# Autodesk Inventor assembly: Rail_AssemblyV2_0
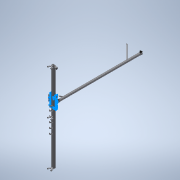
[picture p0: Inventor's stored thumbnail of the model, 180x180]
Saved by Autodesk Inventor 2021 (Build 250183000, 183)
## iProperties
Created: 2021-01-25
Part Number: Rail_AssemblyV2_0
Document SubType Name: Assembly
Designer: Jorian Brusind
Mass: 3786.54 g
Surface Area: 19508.5 cm^2
Volume: 2323.9 cm^3
Density: 1.62939 g/cm^3
Author: Jorian Brusind
## Documents named in this file (30)
- C:\Users\Jorian Brusind\Documents\GitHub\PersonalProjects\HyperRail\Inventor Files\Rail_AssemblyV2_0.iam
- C:\Users\Jorian Brusind\Documents\GitHub\PersonalProjects\Inventor Projects\Useful models\NEMA_Steppers\NEMA23\23HS8430B.ipt
- C:\Users\Jorian Brusind\Documents\GitHub\PersonalProjects\HyperRail\Inventor Files\2804S_NEMA2115_1Gearbox.ipt
- C:\Users\Jorian Brusind\Documents\GitHub\PersonalProjects\HyperRail\PCB Files\Integrated Stepper Motor Driver\ExportSTEP\Main.iam
- C:\Users\Jorian Brusind\Documents\GitHub\PersonalProjects\HyperRail\Inventor Files\NEMA23_Shroud.ipt
- C:\Users\Jorian Brusind\Documents\GitHub\PersonalProjects\Inventor Projects\Useful models\8020_Sets\IPT_20_Series\IPT_20_Series\20-4040_2m.ipt
- C:\Users\Jorian Brusind\Documents\GitHub\PersonalProjects\HyperRail\Inventor Files\98952A059_ALUM MALE-FEM THRDED HEX STANDOFF.ipt
- C:\Users\Jorian Brusind\Documents\GitHub\PersonalProjects\HyperRail\Inventor Files\95783A039_NYLON 6-6 MALE-FEM THRDED HEX STANDOFF.ipt
- C:\Users\Jorian Brusind\Documents\GitHub\PersonalProjects\HyperRail\Inventor Files\Integrated_Stepper_NEMA23_Mount.ipt
- C:\Users\Jorian Brusind\Documents\GitHub\PersonalProjects\Inventor Projects\Useful models\8020_Sets\IPT_40_Series\Extra_40_Series\HFS5-4060-4000\HFS5-4060-2125.ipt
- C:\Users\Jorian Brusind\Documents\GitHub\PersonalProjects\Inventor Projects\Useful models\8020_Sets\AIS2018\20-2568_d.iam
- C:\Users\Jorian Brusind\Documents\GitHub\PersonalProjects\HyperRail\Inventor Files\5mm_bore_10mm_width_idlepulley.ipt
- C:\Users\Jorian Brusind\Documents\GitHub\PersonalProjects\HyperRail\Inventor Files\Tape_Belt_Layer.ipt
- C:\Users\Jorian Brusind\Documents\GitHub\PersonalProjects\HyperRail\Inventor Files\SDP_sdpsi_a_6a55m028df0912\SDP_sdpsi_a_6a55m028df0912.ipt
- C:\Users\Jorian Brusind\Documents\GitHub\PersonalProjects\HyperRail\Inventor Files\SDP_sdpsi_a_6r25mc250\SDP_sdpsi_a_6r25mc1000.ipt
- C:\Users\Jorian Brusind\Documents\GitHub\PersonalProjects\HyperRail\Inventor Files\Cable_Guide_Holder.ipt
- C:\Users\Jorian Brusind\Documents\GitHub\PersonalProjects\HyperRail\Inventor Files\Carriage_Assembly.iam
- C:\Users\Jorian Brusind\Documents\GitHub\PersonalProjects\HyperRail\Inventor Files\NEMA23_StepperonlineMount.ipt
- C:\Users\Jorian Brusind\Documents\GitHub\PersonalProjects\HyperRail\Inventor Files\59145_Sensor.ipt
- C:\Users\Jorian Brusind\Documents\GitHub\PersonalProjects\HyperRail\Inventor Files\RightAngle_SideBracket.ipt
- C:\Users\Jorian Brusind\Documents\GitHub\PersonalProjects\HyperRail\Inventor Files\RightAngle_PulleySupport.ipt
- C:\Users\Jorian Brusind\Documents\GitHub\PersonalProjects\HyperRail\Inventor Files\MagnetHolder.ipt
- C:\Users\Jorian Brusind\Documents\GitHub\PersonalProjects\HyperRail\Inventor Files\MagnetActuatorHolder.ipt
- C:\Users\Jorian Brusind\Documents\GitHub\PersonalProjects\HyperRail\Inventor Files\59145_Actuator.ipt
- C:\Users\Jorian Brusind\Documents\GitHub\PersonalProjects\HyperRail\Inventor Files\Bottom_Foot_Assembly.iam
- C:\Users\Jorian Brusind\Documents\GitHub\PersonalProjects\Inventor Projects\Useful models\Metric bolt\Bolt M5 8mm.ipt
- C:\Users\Jorian Brusind\Documents\GitHub\PersonalProjects\Inventor Projects\Useful models\Metric bolt\Bolt M5 12mm.ipt
- C:\Users\Jorian Brusind\Documents\GitHub\PersonalProjects\Inventor Projects\Useful models\Metric bolt\Bolt M5 25mm.ipt
- C:\Users\Jorian Brusind\Documents\GitHub\PersonalProjects\Inventor Projects\Useful models\Metric bolt\Bolt M4 10mm.ipt
- C:\Users\Jorian Brusind\Documents\GitHub\PersonalProjects\HyperRail\Inventor Files\RightAngle_Bracket_60mm.ipt
## Components (79 placed, 29 different names)
1. 23HS8430B:1 — Mate:127, Angle:3, Mate:158, Mate:177, Mate:179, Mate:180, Mate:181, Mate:182, Mate:183, Mate:184, Mate:185, Mate:264, Mate:265, Mate:295, Angle:5, Angle:6
2. 2804S_NEMA2115_1Gearbox:1 — Mate:127, Angle:3, Mate:158, Flush:86, Mate:336, Flush:126, Mate:370, Mate:371
3. Main:1 [sub-assembly] — Mate:291, Mate:292, Mate:293
4. 20-4040_2m:2 — Flush:123, Mate:322, Mate:323, Mate:354, Flush:143, Flush:156, Mate:375, Flush:158, Mate:377, Mate:378, Flush:160, Flush:161, Flush:163, Flush:189, Mate:420, Flush:190, Mate:474
5. NEMA23_Shroud:1 — Mate:264, Mate:265, Flush:86, Angle:7, Mate:452, Mate:453, Mate:454, Mate:455, Mate:456, Mate:457, Mate:458, Mate:459
6. 98952A059_ALUM MALE-FEM THRDED HEX STANDOFF:1 — Mate:180, Mate:181, Mate:186, Mate:191
7. 98952A059_ALUM MALE-FEM THRDED HEX STANDOFF:2 — Mate:184, Mate:185, Mate:189, Mate:192
8. 98952A059_ALUM MALE-FEM THRDED HEX STANDOFF:3 — Mate:177, Mate:179, Mate:187, Mate:190
9. 98952A059_ALUM MALE-FEM THRDED HEX STANDOFF:4 — Mate:182, Mate:183, Mate:188, Mate:193
10. 95783A039_NYLON 6-6 MALE-FEM THRDED HEX STANDOFF:1 — Mate:188, Mate:193
11. 95783A039_NYLON 6-6 MALE-FEM THRDED HEX STANDOFF:2 — Mate:186, Mate:191, Mate:369
12. 95783A039_NYLON 6-6 MALE-FEM THRDED HEX STANDOFF:3 — Mate:187, Mate:190
13. 95783A039_NYLON 6-6 MALE-FEM THRDED HEX STANDOFF:4 — Mate:189, Mate:192
14. HFS5-4060-2125:1 — Mate:277, Mate:278, Mate:279, Mate:280, Mate:332, Mate:333, Mate:344, Flush:132, Flush:133, Mate:353, Mate:366, Mate:413, Flush:179, Mate:418, Mate:428, Flush:195, Flush:196, Mate:431, Flush:197, Flush:198, Mate:494, Mate:495
15. Integrated_Stepper_NEMA23_Mount:1 — Mate:291, Mate:292, Mate:293, Mate:295, Mate:360, Mate:361, Mate:362, Mate:363, Mate:364, Mate:369, Angle:5, Angle:6
16. 20-2568_d:1 [sub-assembly] — Flush:123, Mate:322, Mate:323
17. 5mm_bore_10mm_width_idlepulley:2 — Mate:421, Mate:422, Mate:446, Mate:447
18. Tape_Belt_Layer:1 — Mate:332, Mate:333
19. SDP_sdpsi_a_6a55m028df0912:1 — Mate:336, Flush:126, Flush:191
20. SDP_sdpsi_a_6r25mc1000:1 — Flush:130, Mate:343, Flush:131, Mate:344, Flush:132, Flush:133
21. SDP_sdpsi_a_6r25mc1000:2 — Flush:130, Mate:343, Flush:131
22. Carriage_Assembly:1 [sub-assembly] — Mate:353, Mate:354, Flush:143, Mate:366, Mate:372, Flush:153, Flush:157, Flush:159, Flush:189, Flush:191, Mate:427, Flush:193, Flush:194, Mate:460, Mate:463, Mate:475, Mate:477, Mate:494, Mate:495
23. 98952A059_ALUM MALE-FEM THRDED HEX STANDOFF:5 — Mate:360, Flush:151, Flush:152
24. 98952A059_ALUM MALE-FEM THRDED HEX STANDOFF:6 — Mate:361, Flush:152
25. 98952A059_ALUM MALE-FEM THRDED HEX STANDOFF:7 — Mate:362, Mate:364, Flush:150, Flush:151
26. 98952A059_ALUM MALE-FEM THRDED HEX STANDOFF:8 — Mate:363, Flush:150
27. NEMA23_StepperonlineMount:1 — Mate:370, Mate:371, Angle:7, Mate:372, Flush:153, Mate:461, Mate:462, Mate:464, Mate:465
28. 59145_Sensor:1 — Mate:425, Mate:426, Angle:8
29. RightAngle_SideBracket:1 — Mate:375, Flush:158, Flush:159, Mate:476, Mate:478, Mate:479, Mate:480, Mate:481, Mate:482, Mate:483, Mate:484, Mate:485
30. RightAngle_SideBracket:2 — Flush:156, Flush:157, Mate:473, Mate:474, Mate:486, Mate:487, Mate:488, Mate:489, Mate:490, Mate:491, Mate:492, Mate:493
31. RightAngle_SideBracket:3 — Mate:378, Flush:160, Flush:162, Flush:163, Mate:438, Mate:439, Mate:440, Mate:441, Mate:442, Mate:443
32. RightAngle_SideBracket:4 — Mate:377, Flush:161, Flush:162, Mate:432, Mate:433, Mate:434, Mate:435, Mate:436, Mate:437
33. Cable_Guide_Holder:1 — Mate:413, Flush:179, Flush:188, Mate:419
34. Cable_Guide_Holder:2 — Mate:414, Flush:180, Flush:181
35. Cable_Guide_Holder:3 — Mate:414, Flush:180, Flush:181, Flush:182, Flush:183, Flush:186, Flush:187, Mate:415
36. Cable_Guide_Holder:4 — Flush:182, Flush:187, Mate:415, Mate:416
37. Cable_Guide_Holder:5 — Flush:183, Flush:184, Flush:185, Flush:186, Mate:417, Mate:418, Flush:188
38. Cable_Guide_Holder:6 — Flush:184, Flush:185, Mate:416, Mate:417, Mate:419
39. RightAngle_PulleySupport:1 — Mate:420, Flush:190, Mate:421, Mate:422, Mate:444, Mate:445
40. MagnetHolder:1 — Mate:425, Mate:426, Mate:427, Flush:193, Angle:8, Flush:194
41. MagnetActuatorHolder:1 — Mate:428, Flush:195, Flush:196, Mate:429, Angle:9, Mate:430, Mate:448, Mate:449, Mate:450, Mate:451
42. 59145_Actuator:1 — Mate:429, Angle:9, Mate:430
43. Bolt M5 8mm:1 — Mate:434, Flush:199, Flush:200, Flush:201, Flush:202, Mate:437
44. Bolt M5 8mm:2 — Mate:432, Flush:201
45. Bolt M5 8mm:3 — Mate:435, Flush:199
46. Bolt M5 8mm:4 — Mate:433, Flush:202
47. Bolt M5 8mm:5 — Mate:442, Flush:206
48. Bolt M5 8mm:6 — Mate:440, Flush:204
49. Bolt M5 8mm:7 — Mate:439, Flush:203, Flush:204, Flush:205, Flush:206, Mate:443
50. Bolt M5 8mm:8 — Mate:438, Flush:203
51. Bolt M5 8mm:9 — Mate:441, Flush:205
52. Bolt M5 8mm:10 — Mate:436, Flush:200
53. Bolt M5 12mm:1 — Mate:444, Mate:445
54. Bolt M5 25mm:1 — Mate:446, Mate:447
55. Bolt M5 12mm:2 — Mate:448, Mate:450
56. Bolt M5 12mm:3 — Mate:449, Mate:451
57. Bolt M4 10mm:1 — Mate:453, Mate:456
58. Bolt M4 10mm:2 — Mate:454, Mate:459
59. Bolt M4 10mm:3 — Mate:455, Mate:458
60. Bolt M4 10mm:4 — Mate:452, Mate:457
61. RightAngle_Bracket_60mm:1 — Mate:460, Mate:461, Mate:464, Mate:468, Mate:469, Mate:470, Mate:471
62. RightAngle_Bracket_60mm:2 — Mate:462, Mate:463, Mate:465, Mate:466, Mate:467, Mate:472
63. Bolt M5 12mm:4 — Mate:469, Mate:471
64. Bolt M5 12mm:5 — Mate:468, Mate:470
65. Bolt M5 12mm:6 — Mate:467
66. Bolt M5 12mm:7 — Mate:466, Mate:472
67. Bolt M5 12mm:8 — Mate:473, Mate:475
68. Bolt M5 12mm:9 — Mate:476, Mate:477
69. Bolt M5 8mm:11 — Mate:478, Mate:483
70. Bolt M5 8mm:12 — Mate:479, Mate:482
71. Bolt M5 8mm:13 — Mate:480, Mate:484
72. Bolt M5 8mm:14 — Mate:481, Mate:485
73. Bolt M5 8mm:15 — Mate:486, Mate:492
74. Bolt M5 8mm:16 — Mate:489, Mate:490
75. Bolt M5 8mm:17 — Mate:487, Mate:491
76. Bolt M5 8mm:18 — Mate:488, Mate:493
77. Bottom_Foot_Assembly:1 [sub-assembly] — Mate:431, Flush:197, Flush:198
78. Bottom_Foot_Assembly:2 [sub-assembly]
79. Bottom_Foot_Assembly:3 [sub-assembly]
## Component patterns: (3 elements, first: Bottom_Foot_Assembly:1)
## Relationships (184: Mate 131, Flush 47, Angle 6)
- Mate:127: 23HS8430B:1 ↔ 2804S_NEMA2115_1Gearbox:1
- Angle:3 (0 deg): 23HS8430B:1 ↔ 2804S_NEMA2115_1Gearbox:1
- Mate:158: 23HS8430B:1 ↔ 2804S_NEMA2115_1Gearbox:1
- Mate:177: 23HS8430B:1 ↔ 98952A059_ALUM MALE-FEM THRDED HEX STANDOFF:3
- Mate:179: 23HS8430B:1 ↔ 98952A059_ALUM MALE-FEM THRDED HEX STANDOFF:3
- Mate:180: 23HS8430B:1 ↔ 98952A059_ALUM MALE-FEM THRDED HEX STANDOFF:1
- Mate:181: 23HS8430B:1 ↔ 98952A059_ALUM MALE-FEM THRDED HEX STANDOFF:1
- Mate:182: 23HS8430B:1 ↔ 98952A059_ALUM MALE-FEM THRDED HEX STANDOFF:4
- Mate:183: 23HS8430B:1 ↔ 98952A059_ALUM MALE-FEM THRDED HEX STANDOFF:4
- Mate:184: 23HS8430B:1 ↔ 98952A059_ALUM MALE-FEM THRDED HEX STANDOFF:2
- Mate:185: 23HS8430B:1 ↔ 98952A059_ALUM MALE-FEM THRDED HEX STANDOFF:2
- Mate:186: 98952A059_ALUM MALE-FEM THRDED HEX STANDOFF:1 ↔ 95783A039_NYLON 6-6 MALE-FEM THRDED HEX STANDOFF:2
- Mate:187: 98952A059_ALUM MALE-FEM THRDED HEX STANDOFF:3 ↔ 95783A039_NYLON 6-6 MALE-FEM THRDED HEX STANDOFF:3
- Mate:188: 98952A059_ALUM MALE-FEM THRDED HEX STANDOFF:4 ↔ 95783A039_NYLON 6-6 MALE-FEM THRDED HEX STANDOFF:1
- Mate:189: 98952A059_ALUM MALE-FEM THRDED HEX STANDOFF:2 ↔ 95783A039_NYLON 6-6 MALE-FEM THRDED HEX STANDOFF:4
- Mate:190: 98952A059_ALUM MALE-FEM THRDED HEX STANDOFF:3 ↔ 95783A039_NYLON 6-6 MALE-FEM THRDED HEX STANDOFF:3
- Mate:191: 98952A059_ALUM MALE-FEM THRDED HEX STANDOFF:1 ↔ 95783A039_NYLON 6-6 MALE-FEM THRDED HEX STANDOFF:2
- Mate:192: 98952A059_ALUM MALE-FEM THRDED HEX STANDOFF:2 ↔ 95783A039_NYLON 6-6 MALE-FEM THRDED HEX STANDOFF:4
- Mate:193: 98952A059_ALUM MALE-FEM THRDED HEX STANDOFF:4 ↔ 95783A039_NYLON 6-6 MALE-FEM THRDED HEX STANDOFF:1
- Mate:264 (1 mm): 23HS8430B:1 ↔ NEMA23_Shroud:1
- Mate:265 (1 mm): 23HS8430B:1 ↔ NEMA23_Shroud:1
- Flush:86: 2804S_NEMA2115_1Gearbox:1 ↔ NEMA23_Shroud:1
- Mate:277: HFS5-4060-2125:1
- Mate:278: HFS5-4060-2125:1
- Mate:279: HFS5-4060-2125:1
- Mate:280: HFS5-4060-2125:1
- Mate:291: Main:1 ↔ Integrated_Stepper_NEMA23_Mount:1
- Mate:292: Main:1 ↔ Integrated_Stepper_NEMA23_Mount:1
- Mate:293: Main:1 ↔ Integrated_Stepper_NEMA23_Mount:1
- Mate:295: 23HS8430B:1 ↔ Integrated_Stepper_NEMA23_Mount:1
- Flush:123: 20-4040_2m:2 ↔ 20-2568_d:1
- Mate:322 (-2 mm): 20-4040_2m:2 ↔ 20-2568_d:1
- Mate:323: 20-4040_2m:2 ↔ 20-2568_d:1
- Mate:332: HFS5-4060-2125:1 ↔ Tape_Belt_Layer:1
- Mate:333 (1 mm): HFS5-4060-2125:1 ↔ Tape_Belt_Layer:1
- Mate:336: 2804S_NEMA2115_1Gearbox:1 ↔ SDP_sdpsi_a_6a55m028df0912:1
- Flush:126: 2804S_NEMA2115_1Gearbox:1 ↔ SDP_sdpsi_a_6a55m028df0912:1
- Flush:130: SDP_sdpsi_a_6r25mc1000:1 ↔ SDP_sdpsi_a_6r25mc1000:2
- Mate:343: SDP_sdpsi_a_6r25mc1000:1 ↔ SDP_sdpsi_a_6r25mc1000:2
- Flush:131: SDP_sdpsi_a_6r25mc1000:1 ↔ SDP_sdpsi_a_6r25mc1000:2
- Mate:344 (1 mm): HFS5-4060-2125:1 ↔ SDP_sdpsi_a_6r25mc1000:1
- Flush:132: HFS5-4060-2125:1 ↔ SDP_sdpsi_a_6r25mc1000:1
- Flush:133: HFS5-4060-2125:1 ↔ SDP_sdpsi_a_6r25mc1000:1
- Mate:353 (6 mm): HFS5-4060-2125:1 ↔ Carriage_Assembly:1
- Mate:354: 20-4040_2m:2 ↔ Carriage_Assembly:1
- Flush:143: 20-4040_2m:2 ↔ Carriage_Assembly:1
- Mate:360: Integrated_Stepper_NEMA23_Mount:1 ↔ 98952A059_ALUM MALE-FEM THRDED HEX STANDOFF:5
- Mate:361: Integrated_Stepper_NEMA23_Mount:1 ↔ 98952A059_ALUM MALE-FEM THRDED HEX STANDOFF:6
- Mate:362: Integrated_Stepper_NEMA23_Mount:1 ↔ 98952A059_ALUM MALE-FEM THRDED HEX STANDOFF:7
- Mate:363: Integrated_Stepper_NEMA23_Mount:1 ↔ 98952A059_ALUM MALE-FEM THRDED HEX STANDOFF:8
- Mate:364: Integrated_Stepper_NEMA23_Mount:1 ↔ 98952A059_ALUM MALE-FEM THRDED HEX STANDOFF:7
- Flush:150: 98952A059_ALUM MALE-FEM THRDED HEX STANDOFF:7 ↔ 98952A059_ALUM MALE-FEM THRDED HEX STANDOFF:8
- Flush:151: 98952A059_ALUM MALE-FEM THRDED HEX STANDOFF:5 ↔ 98952A059_ALUM MALE-FEM THRDED HEX STANDOFF:7
- Flush:152: 98952A059_ALUM MALE-FEM THRDED HEX STANDOFF:5 ↔ 98952A059_ALUM MALE-FEM THRDED HEX STANDOFF:6
- Mate:366 (26.5 mm): HFS5-4060-2125:1 ↔ Carriage_Assembly:1
- Mate:369: 95783A039_NYLON 6-6 MALE-FEM THRDED HEX STANDOFF:2 ↔ Integrated_Stepper_NEMA23_Mount:1
- Angle:5 (0 deg): 23HS8430B:1 ↔ Integrated_Stepper_NEMA23_Mount:1
- Angle:6 (0 deg): 23HS8430B:1 ↔ Integrated_Stepper_NEMA23_Mount:1
- Mate:370: 2804S_NEMA2115_1Gearbox:1 ↔ NEMA23_StepperonlineMount:1
- Mate:371: 2804S_NEMA2115_1Gearbox:1 ↔ NEMA23_StepperonlineMount:1
- Angle:7 (0 deg): NEMA23_Shroud:1 ↔ NEMA23_StepperonlineMount:1
- Mate:372: Carriage_Assembly:1 ↔ NEMA23_StepperonlineMount:1
- Flush:153 (-11.25 mm): Carriage_Assembly:1 ↔ NEMA23_StepperonlineMount:1
- Flush:156: 20-4040_2m:2 ↔ RightAngle_SideBracket:2
- Flush:157: Carriage_Assembly:1 ↔ RightAngle_SideBracket:2
- Mate:375: 20-4040_2m:2 ↔ RightAngle_SideBracket:1
- Flush:158: 20-4040_2m:2 ↔ RightAngle_SideBracket:1
- Flush:159: Carriage_Assembly:1 ↔ RightAngle_SideBracket:1
- Mate:377: 20-4040_2m:2 ↔ RightAngle_SideBracket:4
- Mate:378: 20-4040_2m:2 ↔ RightAngle_SideBracket:3
- Flush:160: 20-4040_2m:2 ↔ RightAngle_SideBracket:3
- Flush:161: 20-4040_2m:2 ↔ RightAngle_SideBracket:4
- Flush:162: RightAngle_SideBracket:3 ↔ RightAngle_SideBracket:4
- Flush:163 (-20 mm): 20-4040_2m:2 ↔ RightAngle_SideBracket:3
- Mate:413: HFS5-4060-2125:1 ↔ Cable_Guide_Holder:1
- Flush:179: HFS5-4060-2125:1 ↔ Cable_Guide_Holder:1
- Mate:414 (100 mm): Cable_Guide_Holder:2 ↔ Cable_Guide_Holder:3
- Flush:180: Cable_Guide_Holder:2 ↔ Cable_Guide_Holder:3
- Flush:181: Cable_Guide_Holder:2 ↔ Cable_Guide_Holder:3
- Flush:182: Cable_Guide_Holder:3 ↔ Cable_Guide_Holder:4
- Flush:183: Cable_Guide_Holder:3 ↔ Cable_Guide_Holder:5
- Flush:184: Cable_Guide_Holder:5 ↔ Cable_Guide_Holder:6
- Flush:185: Cable_Guide_Holder:5 ↔ Cable_Guide_Holder:6
- Flush:186: Cable_Guide_Holder:3 ↔ Cable_Guide_Holder:5
- Flush:187: Cable_Guide_Holder:3 ↔ Cable_Guide_Holder:4
- Mate:415 (100 mm): Cable_Guide_Holder:3 ↔ Cable_Guide_Holder:4
- Mate:416 (100 mm): Cable_Guide_Holder:4 ↔ Cable_Guide_Holder:6
- Mate:417 (100 mm): Cable_Guide_Holder:5 ↔ Cable_Guide_Holder:6
- Mate:418: HFS5-4060-2125:1 ↔ Cable_Guide_Holder:5
- Flush:188: Cable_Guide_Holder:1 ↔ Cable_Guide_Holder:5
- Mate:419 (200 mm): Cable_Guide_Holder:1 ↔ Cable_Guide_Holder:6
- Flush:189: 20-4040_2m:2 ↔ Carriage_Assembly:1
- Mate:420: 20-4040_2m:2 ↔ RightAngle_PulleySupport:1
- Flush:190: 20-4040_2m:2 ↔ RightAngle_PulleySupport:1
- Mate:421: 5mm_bore_10mm_width_idlepulley:2 ↔ RightAngle_PulleySupport:1
- Mate:422 (5 mm): 5mm_bore_10mm_width_idlepulley:2 ↔ RightAngle_PulleySupport:1
- Flush:191: SDP_sdpsi_a_6a55m028df0912:1 ↔ Carriage_Assembly:1
- Mate:425: 59145_Sensor:1 ↔ MagnetHolder:1
- Mate:426: 59145_Sensor:1 ↔ MagnetHolder:1
- Mate:427: Carriage_Assembly:1 ↔ MagnetHolder:1
- Flush:193: Carriage_Assembly:1 ↔ MagnetHolder:1
- Angle:8 (0 deg): 59145_Sensor:1 ↔ MagnetHolder:1
- Flush:194: Carriage_Assembly:1 ↔ MagnetHolder:1
- Mate:428: HFS5-4060-2125:1 ↔ MagnetActuatorHolder:1
- Flush:195: HFS5-4060-2125:1 ↔ MagnetActuatorHolder:1
- Flush:196: HFS5-4060-2125:1 ↔ MagnetActuatorHolder:1
- Mate:429: MagnetActuatorHolder:1 ↔ 59145_Actuator:1
- Angle:9 (0 deg): MagnetActuatorHolder:1 ↔ 59145_Actuator:1
- Mate:430: MagnetActuatorHolder:1 ↔ 59145_Actuator:1
- Mate:431: HFS5-4060-2125:1 ↔ Bottom_Foot_Assembly:1
- Flush:197 (8 mm): HFS5-4060-2125:1 ↔ Bottom_Foot_Assembly:1
- Flush:198: HFS5-4060-2125:1 ↔ Bottom_Foot_Assembly:1
- Mate:432: RightAngle_SideBracket:4 ↔ Bolt M5 8mm:2
- Mate:433: RightAngle_SideBracket:4 ↔ Bolt M5 8mm:4
- Mate:434: RightAngle_SideBracket:4 ↔ Bolt M5 8mm:1
- Mate:435: RightAngle_SideBracket:4 ↔ Bolt M5 8mm:3
- Mate:436: RightAngle_SideBracket:4 ↔ Bolt M5 8mm:10
- Flush:199: Bolt M5 8mm:1 ↔ Bolt M5 8mm:3
- Flush:200: Bolt M5 8mm:1 ↔ Bolt M5 8mm:10
- Flush:201: Bolt M5 8mm:1 ↔ Bolt M5 8mm:2
- Flush:202: Bolt M5 8mm:1 ↔ Bolt M5 8mm:4
- Mate:437: RightAngle_SideBracket:4 ↔ Bolt M5 8mm:1
- Mate:438: RightAngle_SideBracket:3 ↔ Bolt M5 8mm:8
- Mate:439: RightAngle_SideBracket:3 ↔ Bolt M5 8mm:7
- Mate:440: RightAngle_SideBracket:3 ↔ Bolt M5 8mm:6
- Mate:441: RightAngle_SideBracket:3 ↔ Bolt M5 8mm:9
- Mate:442: RightAngle_SideBracket:3 ↔ Bolt M5 8mm:5
- Flush:203: Bolt M5 8mm:7 ↔ Bolt M5 8mm:8
- Flush:204: Bolt M5 8mm:6 ↔ Bolt M5 8mm:7
- Flush:205: Bolt M5 8mm:7 ↔ Bolt M5 8mm:9
- Flush:206: Bolt M5 8mm:5 ↔ Bolt M5 8mm:7
- Mate:443: RightAngle_SideBracket:3 ↔ Bolt M5 8mm:7
- Mate:444: RightAngle_PulleySupport:1 ↔ Bolt M5 12mm:1
- Mate:445: RightAngle_PulleySupport:1 ↔ Bolt M5 12mm:1
- Mate:446: 5mm_bore_10mm_width_idlepulley:2 ↔ Bolt M5 25mm:1
- Mate:447: 5mm_bore_10mm_width_idlepulley:2 ↔ Bolt M5 25mm:1
- Mate:448: MagnetActuatorHolder:1 ↔ Bolt M5 12mm:2
- Mate:449: MagnetActuatorHolder:1 ↔ Bolt M5 12mm:3
- Mate:450: MagnetActuatorHolder:1 ↔ Bolt M5 12mm:2
- Mate:451: MagnetActuatorHolder:1 ↔ Bolt M5 12mm:3
- Mate:452: NEMA23_Shroud:1 ↔ Bolt M4 10mm:4
- Mate:453: NEMA23_Shroud:1 ↔ Bolt M4 10mm:1
- Mate:454: NEMA23_Shroud:1 ↔ Bolt M4 10mm:2
- Mate:455: NEMA23_Shroud:1 ↔ Bolt M4 10mm:3
- Mate:456: NEMA23_Shroud:1 ↔ Bolt M4 10mm:1
- Mate:457: NEMA23_Shroud:1 ↔ Bolt M4 10mm:4
- Mate:458: NEMA23_Shroud:1 ↔ Bolt M4 10mm:3
- Mate:459: NEMA23_Shroud:1 ↔ Bolt M4 10mm:2
- Mate:460: Carriage_Assembly:1 ↔ RightAngle_Bracket_60mm:1
- Mate:461: NEMA23_StepperonlineMount:1 ↔ RightAngle_Bracket_60mm:1
- Mate:462: NEMA23_StepperonlineMount:1 ↔ RightAngle_Bracket_60mm:2
- Mate:463: Carriage_Assembly:1 ↔ RightAngle_Bracket_60mm:2
- Mate:464 (3 mm): NEMA23_StepperonlineMount:1 ↔ RightAngle_Bracket_60mm:1
- Mate:465 (3 mm): NEMA23_StepperonlineMount:1 ↔ RightAngle_Bracket_60mm:2
- Mate:466: RightAngle_Bracket_60mm:2 ↔ Bolt M5 12mm:7
- Mate:467: RightAngle_Bracket_60mm:2 ↔ Bolt M5 12mm:6
- Mate:468: RightAngle_Bracket_60mm:1 ↔ Bolt M5 12mm:5
- Mate:469: RightAngle_Bracket_60mm:1 ↔ Bolt M5 12mm:4
- Mate:470: RightAngle_Bracket_60mm:1 ↔ Bolt M5 12mm:5
- Mate:471: RightAngle_Bracket_60mm:1 ↔ Bolt M5 12mm:4
- Mate:472: RightAngle_Bracket_60mm:2 ↔ Bolt M5 12mm:7
- Mate:473: RightAngle_SideBracket:2 ↔ Bolt M5 12mm:8
- Mate:474: 20-4040_2m:2 ↔ RightAngle_SideBracket:2
- Mate:475: Carriage_Assembly:1 ↔ Bolt M5 12mm:8
- Mate:476: RightAngle_SideBracket:1 ↔ Bolt M5 12mm:9
- Mate:477: Carriage_Assembly:1 ↔ Bolt M5 12mm:9
- Mate:478: RightAngle_SideBracket:1 ↔ Bolt M5 8mm:11
- Mate:479: RightAngle_SideBracket:1 ↔ Bolt M5 8mm:12
- Mate:480: RightAngle_SideBracket:1 ↔ Bolt M5 8mm:13
- Mate:481: RightAngle_SideBracket:1 ↔ Bolt M5 8mm:14
- Mate:482: RightAngle_SideBracket:1 ↔ Bolt M5 8mm:12
- Mate:483: RightAngle_SideBracket:1 ↔ Bolt M5 8mm:11
- Mate:484: RightAngle_SideBracket:1 ↔ Bolt M5 8mm:13
- Mate:485: RightAngle_SideBracket:1 ↔ Bolt M5 8mm:14
- Mate:486: RightAngle_SideBracket:2 ↔ Bolt M5 8mm:15
- Mate:487: RightAngle_SideBracket:2 ↔ Bolt M5 8mm:17
- Mate:488: RightAngle_SideBracket:2 ↔ Bolt M5 8mm:18
- Mate:489: RightAngle_SideBracket:2 ↔ Bolt M5 8mm:16
- Mate:490: RightAngle_SideBracket:2 ↔ Bolt M5 8mm:16
- Mate:491: RightAngle_SideBracket:2 ↔ Bolt M5 8mm:17
- Mate:492: RightAngle_SideBracket:2 ↔ Bolt M5 8mm:15
- Mate:493: RightAngle_SideBracket:2 ↔ Bolt M5 8mm:18
- Mate:494 (12 mm): HFS5-4060-2125:1 ↔ Carriage_Assembly:1
- Mate:495 (12 mm): HFS5-4060-2125:1 ↔ Carriage_Assembly:1
